# Autodesk Inventor assembly: Sensorboard
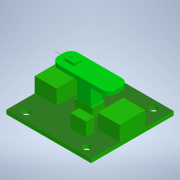
[picture p0: Inventor's stored thumbnail of the model, 180x180]
Saved by Autodesk Inventor 2020.2 (Build 242310000, 310)
## iProperties
Created: 2020-02-12
Part Number: Sensorboard
Document SubType Name: Assembly
Designer: Max
Author: Max
## Documents named in this file (3)
- D:\Eigene Dateien\Dokumente\SynologyDrive\Uni\Studienarbeit\Eigene Inhalte\GehäuseCad\Standardteile\Mirofonboard\Sensorboard.iam
- D:\Eigene Dateien\Dokumente\SynologyDrive\Uni\Studienarbeit\Eigene Inhalte\GehäuseCad\Standardteile\Mirofonboard\Prozessorboard.ipt
- D:\Eigene Dateien\Dokumente\SynologyDrive\Uni\Studienarbeit\Eigene Inhalte\GehäuseCad\Standardteile\Mirofonboard\Mikrofonboard.ipt
## Components (2 placed, 2 different names)
1. Prozessorboard:1 — Fluchtend:1, Fluchtend:2, Passend:1
2. Mikrofonboard:1 — Fluchtend:1, Fluchtend:2, Passend:1
## Relationships (3: Flush 2, Mate 1)
- Fluchtend:1 [Flush] (0.75 mm): Prozessorboard:1 ↔ Mikrofonboard:1
- Fluchtend:2 [Flush] (0.05 mm): Prozessorboard:1 ↔ Mikrofonboard:1
- Passend:1 [Mate]: Prozessorboard:1 ↔ Mikrofonboard:1
